# Autodesk Inventor assembly: Assembly1
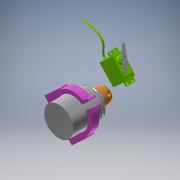
[picture p0: Inventor's stored thumbnail of the model, 180x180]
Saved by Autodesk Inventor 2016 (Build 200138000, 138)
## iProperties
Created: 2016-04-17
Part Number: Assembly1
Document SubType Name: Assembly
Designer: amenoni
Author: amenoni
## Documents named in this file (6)
- Z:\Desarrollo\WetMaths\wetMaths-Arduino\wetMaths\HwDesigns\Assembly1.iam
- Z:\Desarrollo\WetMaths\wetMaths-Arduino\wetMaths\HwDesigns\SprayCan.ipt
- Z:\Desarrollo\WetMaths\wetMaths-Arduino\wetMaths\HwDesigns\Clamp.ipt
- Z:\Desarrollo\WetMaths\wetMaths-Arduino\wetMaths\HwDesigns\CanNozzle.ipt
- Z:\Desarrollo\WetMaths\wetMaths-Arduino\wetMaths\HwDesigns\Futaba S3004.ipt
- Z:\Desarrollo\WetMaths\wetMaths-Arduino\wetMaths\HwDesigns\Servo_arm_np1.ipt
## Components (5 placed, 5 different names)
1. SprayCan:1 — Mate:1, Mate:2, Mate:3
2. Clamp:1 — Mate:1, Flush:1
3. CanNozzle:1 — Mate:2, Mate:3
4. Futaba S3004:1 — Flush:1, Mate:4, Mate:5
5. Servo_arm_np1:1 — Mate:4, Mate:5
## Relationships (6: Mate 5, Flush 1)
- Mate:1: SprayCan:1 ↔ Clamp:1
- Mate:2: SprayCan:1 ↔ CanNozzle:1
- Mate:3 (2.5 mm): SprayCan:1 ↔ CanNozzle:1
- Flush:1: Clamp:1 ↔ Futaba S3004:1
- Mate:4: Futaba S3004:1 ↔ Servo_arm_np1:1
- Mate:5: Futaba S3004:1 ↔ Servo_arm_np1:1
